# Autodesk Inventor assembly: Piston_Bottom_Hinge
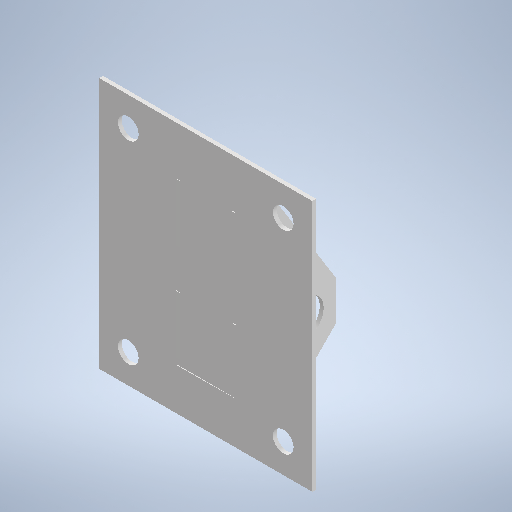
[picture p0: Inventor's stored thumbnail of the model, 512x512]
Saved by Autodesk Inventor 2025.2 (Build 292293000, 293)
## iProperties
Created: 2025-04-08
Part Number: Piston_Bottom_Hinge
Document SubType Name: Assembly
Designer: Victor
Author: Victor
## Documents named in this file (4)
- C:\Users\Victor\Documents\LineFollowerRobot\Anomaly_Detection\Mechanical_Project\Inventor_project\Piston_Bottom_Hinge.iam
- C:\Users\Victor\Documents\LineFollowerRobot\Anomaly_Detection\Mechanical_Project\Inventor_project\Piston_FloorHinge_BasePlate.ipt
- C:\Users\Victor\Documents\LineFollowerRobot\Anomaly_Detection\Mechanical_Project\Inventor_project\Piston_FloorHinge01.ipt
- C:\Users\Victor\Documents\LineFollowerRobot\Anomaly_Detection\Mechanical_Project\Inventor_project\Piston_FloorHinge02.ipt
## Components (4 placed, 3 different names)
1. Piston_FloorHinge_BasePlate:1 — Mate:1, Mate:2, Mate:3
2. Piston_FloorHinge01:1 — Mate:2
3. Piston_FloorHinge01:2 — Mate:3
4. Piston_FloorHinge02:1 — Mate:1
## Relationships (3: Mate 3)
- Mate:1: Piston_FloorHinge_BasePlate:1 ↔ Piston_FloorHinge02:1
- Mate:2: Piston_FloorHinge_BasePlate:1 ↔ Piston_FloorHinge01:1
- Mate:3: Piston_FloorHinge_BasePlate:1 ↔ Piston_FloorHinge01:2
